# Autodesk Inventor assembly: Assembly1.1
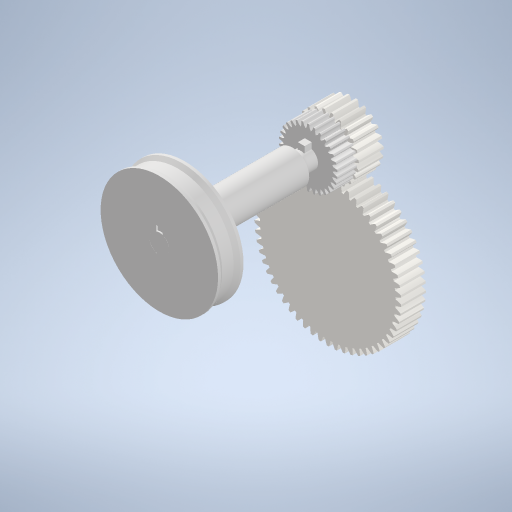
[picture p0: Inventor's stored thumbnail of the model, 512x512]
Saved by Autodesk Inventor 2024 (Build 280153000, 153)
## iProperties
Created: 2024-03-19
Part Number: Assembly1.1
Document SubType Name: Assembly
Designer: manur
Author: manur
## Documents named in this file (6)
- C:\Users\manur\OneDrive\Escritorio\Manuel Fernández\UNIVERSIDAD\semestre actual\Dinámica\Assembly1.1.iam
- C:\Users\manur\Downloads\EJE_CUÑEROS.ipt
- C:\Users\manur\Downloads\ENGRANE.ipt
- C:\Users\manur\Downloads\POLEA.ipt
- C:\Users\manur\Downloads\CUÑA.ipt
- C:\Users\manur\OneDrive\Escritorio\Manuel Fernández\UNIVERSIDAD\semestre actual\Dinámica\Assembly1\Design Accelerator\Spur Gears1.iam
## Components (6 placed, 5 different names)
1. EJE_CUÑEROS:1 — Rigid:1, Mate:1, Mate:2, Cylindrical:1, Flush:1, Rigid:2, Mate:3, Rigid:3, Flush:2, Flush:3, Rotational:1
2. ENGRANE:1 — Cylindrical:1, Flush:1
3. POLEA:1 — Rigid:1, Mate:1, Mate:2
4. CUÑA:1 — Rigid:3, Flush:2, Flush:3
5. CUÑA:2 — Rigid:2, Mate:3
6. Spur Gears:1 [sub-assembly] — Rotational:1
## Relationships (11: WeldJoint 3, Mate 3, Flush 3, CylindricalJoint 1, RevoluteJoint 1)
- Rigid:1 [WeldJoint]: EJE_CUÑEROS:1 ↔ POLEA:1
- Mate:1: EJE_CUÑEROS:1 ↔ POLEA:1
- Mate:2: EJE_CUÑEROS:1 ↔ POLEA:1
- Cylindrical:1: EJE_CUÑEROS:1 ↔ ENGRANE:1
- Flush:1: EJE_CUÑEROS:1 ↔ ENGRANE:1
- Rigid:2 [WeldJoint]: EJE_CUÑEROS:1 ↔ CUÑA:2
- Mate:3: EJE_CUÑEROS:1 ↔ CUÑA:2
- Rigid:3 [WeldJoint]: EJE_CUÑEROS:1 ↔ CUÑA:1
- Flush:2 (-8.001 mm): EJE_CUÑEROS:1 ↔ CUÑA:1
- Flush:3: EJE_CUÑEROS:1 ↔ CUÑA:1
- Rotational:1 [RevoluteJoint]: EJE_CUÑEROS:1 ↔ Spur Gears:1
